# Autodesk Inventor assembly: CE-9.1.5
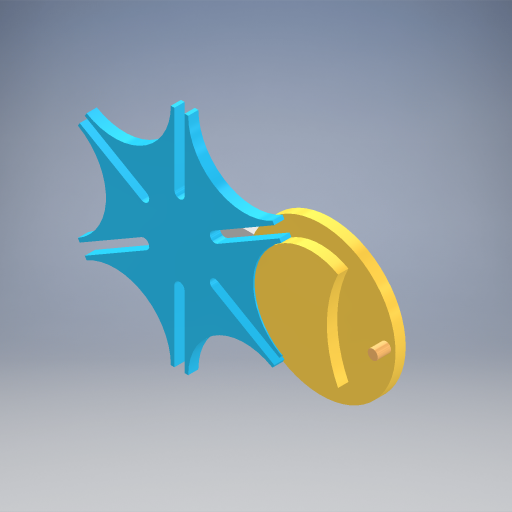
[picture p0: Inventor's stored thumbnail of the model, 512x512]
Saved by Autodesk Inventor 2024 (Build 280153000, 153)
## iProperties
Created: 2024-03-15
Part Number: CE-9.1.5
Document SubType Name: Assembly
Designer: Alex
Author: Alex
## Documents named in this file (4)
- C:\Shared\alex-bartella-schoolwork\4z03\Week 9\CE-9.1.5.iam
- C:\Shared\alex-bartella-schoolwork\4z03\Week 9\STEP\CE-9.1.5 STEP Files\Ground Connector\Ground Connector.ipt
- C:\Shared\alex-bartella-schoolwork\4z03\Week 9\STEP\CE-9.1.5 STEP Files\Input Disk\Input Disk.ipt
- C:\Shared\alex-bartella-schoolwork\4z03\Week 9\STEP\CE-9.1.5 STEP Files\Output Geneva wheel\Output Geneva wheel.ipt
## Components (3 placed, 3 different names)
1. Ground Connector:1 — Flush:1, Flush:2, Flush:3, Mate:1, Mate:2, Mate:3, Mate:5, Angle:1
2. Input Disk:1 — Mate:1, Mate:3, Mate:4
3. Output Geneva wheel:1 — Mate:2, Mate:4
## Relationships (9: Mate 5, Flush 3, Angle 1)
- Flush:1: Ground Connector:1
- Flush:2: Ground Connector:1
- Flush:3: Ground Connector:1
- Mate:1: Ground Connector:1 ↔ Input Disk:1
- Mate:2: Ground Connector:1 ↔ Output Geneva wheel:1
- Mate:3 (1 mm): Ground Connector:1 ↔ Input Disk:1
- Mate:4 (1 mm): Input Disk:1 ↔ Output Geneva wheel:1
- Mate:5: Ground Connector:1
- Angle:1 (0 deg): Ground Connector:1
## Named parameters: Simulation_Timeline = 0
